# Autodesk Inventor assembly: Shock240mm
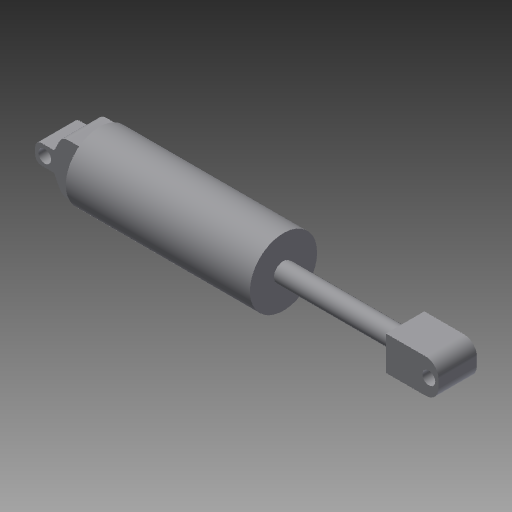
[picture p0: Inventor's stored thumbnail of the model, 512x512]
Saved by Autodesk Inventor 2018 (Build 220112000, 112)
## iProperties
Created: 2018-01-25
Part Number: Shock240mm
Document SubType Name: Assembly
Designer: eroldan
Author: eroldan
## Documents named in this file (3)
- C:\Users\eroldan\Desktop\3dprojects\OpenEmoto\OtherParts\Shock240mm.iam
- C:\Users\eroldan\Desktop\3dprojects\OpenEmoto\OtherParts\ShockBottle_1.ipt
- C:\Users\eroldan\Desktop\3dprojects\OpenEmoto\OtherParts\ShockShaft.ipt
## Components (2 placed, 2 different names)
1. ShockBottle_1:1 — Mate:1, Mate:2, Flush:1
2. ShockShaft:1 — Mate:1, Mate:2, Flush:1
## Relationships (3: Mate 2, Flush 1)
- Mate:1: ShockBottle_1:1 ↔ ShockShaft:1
- Mate:2 (76 mm): ShockBottle_1:1 ↔ ShockShaft:1
- Flush:1: ShockBottle_1:1 ↔ ShockShaft:1
